# Autodesk Inventor assembly: Joining Plate for 4040 Assembly - C
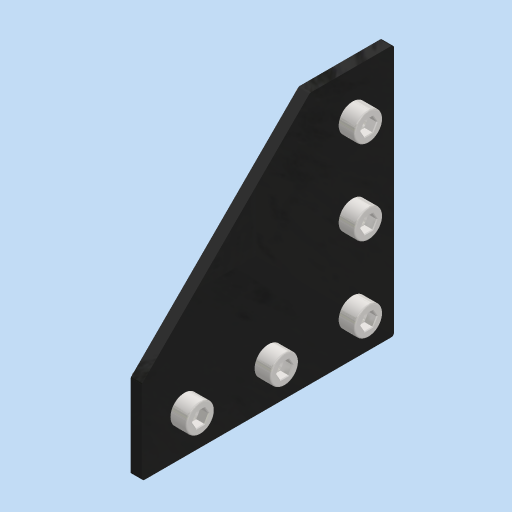
[picture p0: Inventor's stored thumbnail of the model, 512x512]
Saved by Autodesk Inventor 2023.2 (Build 272271000, 271)
## iProperties
Created: 2023-11-20
Part Number: Joining Plate for 4040 Assembly - C
Document SubType Name: Assembly
Designer: Nils Bade
Author: Nils Bade
## Documents named in this file (4)
- C:\Users\nilsb\Documents\Inventor\Projektarbeit-Bade\RatRig_modified\Joining Plate for 4040 Assembly - C.iam
- C:\Users\nilsb\Documents\Inventor\Projektarbeit-Bade\RatRig_Standards\Joining Plate for 3030 - 90 Degree - Black Anodized v2.ipt
- C:\Users\nilsb\Documents\Inventor\Projektarbeit-Bade\Schrauben\Cap Head Screw M6x12 v2.ipt
- C:\Users\nilsb\Documents\Inventor\Projektarbeit-Bade\RatRig_modified\T-NUT - DropIn 4040 SERIES - M6.ipt
## Components (11 placed, 3 different names)
1. Joining Plate for 3030 - 90 Degree - Black Anodized v2:2 — Passend:1, Passend:2, Passend:3, Passend:4, Passend:5, Passend:6, Passend:7, Passend:8, Passend:9, Passend:10, Passend:16, Passend:17, Passend:18, Passend:19, Passend:20
2. Cap Head Screw M6x12 v2:1 — Passend:5, Passend:6, Passend:15
3. Cap Head Screw M6x12 v2:2 — Passend:4, Passend:7, Passend:14
4. Cap Head Screw M6x12 v2:3 — Passend:2, Passend:9, Passend:12
5. Cap Head Screw M6x12 v2:4 — Passend:3, Passend:10, Passend:11
6. Cap Head Screw M6x12 v2:5 — Passend:1, Passend:8, Passend:13
7. T-NUT - DROP IN TYPE FOR 40 SERIES - M6:1 — Passend:15, Winkel:1, Passend:20
8. T-NUT - DROP IN TYPE FOR 40 SERIES - M6:2 — Passend:14, Winkel:2, Passend:19
9. T-NUT - DROP IN TYPE FOR 40 SERIES - M6:3 — Passend:13, Passend:18, Winkel:6
10. T-NUT - DROP IN TYPE FOR 40 SERIES - M6:4 — Passend:12, Winkel:4, Passend:17
11. T-NUT - DROP IN TYPE FOR 40 SERIES - M6:5 — Passend:11, Winkel:5, Passend:16
## Relationships (25: Mate 20, Angle 5)
- Passend:1 [Mate]: Joining Plate for 3030 - 90 Degree - Black Anodized v2:2 ↔ Cap Head Screw M6x12 v2:5
- Passend:2 [Mate]: Joining Plate for 3030 - 90 Degree - Black Anodized v2:2 ↔ Cap Head Screw M6x12 v2:3
- Passend:3 [Mate]: Joining Plate for 3030 - 90 Degree - Black Anodized v2:2 ↔ Cap Head Screw M6x12 v2:4
- Passend:4 [Mate]: Joining Plate for 3030 - 90 Degree - Black Anodized v2:2 ↔ Cap Head Screw M6x12 v2:2
- Passend:5 [Mate]: Joining Plate for 3030 - 90 Degree - Black Anodized v2:2 ↔ Cap Head Screw M6x12 v2:1
- Passend:6 [Mate]: Joining Plate for 3030 - 90 Degree - Black Anodized v2:2 ↔ Cap Head Screw M6x12 v2:1
- Passend:7 [Mate]: Joining Plate for 3030 - 90 Degree - Black Anodized v2:2 ↔ Cap Head Screw M6x12 v2:2
- Passend:8 [Mate]: Joining Plate for 3030 - 90 Degree - Black Anodized v2:2 ↔ Cap Head Screw M6x12 v2:5
- Passend:9 [Mate]: Joining Plate for 3030 - 90 Degree - Black Anodized v2:2 ↔ Cap Head Screw M6x12 v2:3
- Passend:10 [Mate]: Joining Plate for 3030 - 90 Degree - Black Anodized v2:2 ↔ Cap Head Screw M6x12 v2:4
- Passend:11 [Mate]: Cap Head Screw M6x12 v2:4 ↔ T-NUT - DROP IN TYPE FOR 40 SERIES - M6:5
- Passend:12 [Mate]: Cap Head Screw M6x12 v2:3 ↔ T-NUT - DROP IN TYPE FOR 40 SERIES - M6:4
- Passend:13 [Mate]: Cap Head Screw M6x12 v2:5 ↔ T-NUT - DROP IN TYPE FOR 40 SERIES - M6:3
- Passend:14 [Mate]: Cap Head Screw M6x12 v2:2 ↔ T-NUT - DROP IN TYPE FOR 40 SERIES - M6:2
- Passend:15 [Mate]: Cap Head Screw M6x12 v2:1 ↔ T-NUT - DROP IN TYPE FOR 40 SERIES - M6:1
- Winkel:1 [Angle] (0 deg): T-NUT - DROP IN TYPE FOR 40 SERIES - M6:1
- Winkel:2 [Angle] (0 deg): T-NUT - DROP IN TYPE FOR 40 SERIES - M6:2
- Winkel:4 [Angle] (0 deg): T-NUT - DROP IN TYPE FOR 40 SERIES - M6:4
- Winkel:5 [Angle] (0 deg): T-NUT - DROP IN TYPE FOR 40 SERIES - M6:5
- Passend:16 [Mate] (5.5 mm): Joining Plate for 3030 - 90 Degree - Black Anodized v2:2 ↔ T-NUT - DROP IN TYPE FOR 40 SERIES - M6:5
- Passend:17 [Mate] (5.5 mm): Joining Plate for 3030 - 90 Degree - Black Anodized v2:2 ↔ T-NUT - DROP IN TYPE FOR 40 SERIES - M6:4
- Passend:18 [Mate] (5.5 mm): Joining Plate for 3030 - 90 Degree - Black Anodized v2:2 ↔ T-NUT - DROP IN TYPE FOR 40 SERIES - M6:3
- Passend:19 [Mate] (5.5 mm): Joining Plate for 3030 - 90 Degree - Black Anodized v2:2 ↔ T-NUT - DROP IN TYPE FOR 40 SERIES - M6:2
- Passend:20 [Mate] (5.5 mm): Joining Plate for 3030 - 90 Degree - Black Anodized v2:2 ↔ T-NUT - DROP IN TYPE FOR 40 SERIES - M6:1
- Winkel:6 [Angle] (0 deg): T-NUT - DROP IN TYPE FOR 40 SERIES - M6:3
